# Autodesk Inventor assembly: wheel_axle
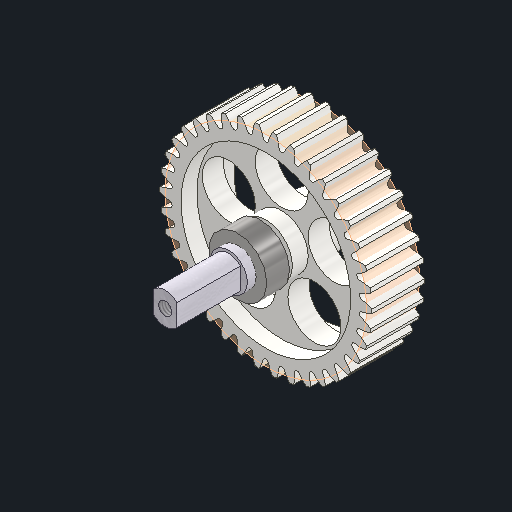
[picture p0: Inventor's stored thumbnail of the model, 512x512]
Saved by Autodesk Inventor 2023 (Build 270158000, 158)
## iProperties
Created: 2024-04-09
Part Number: wheel_axle
Document SubType Name: Assembly
Designer: szymo
Mass: 22 g
Surface Area: 67.2828 cm^2
Volume: 6.31995 cm^3
Density: 3.48104 g/cm^3
Author: szymo
## Documents named in this file (5)
- D:\roboilo\robots\codename wafel - australia\3d_parts\rev4\wheel_axle.iam
- D:\roboilo\robots\codename wafel - australia\3d_parts\rev4\MegaSumo kola zebate 38.ipt
- D:\roboilo\robots\codename wafel - australia\3d_parts\rev4\wal_kola.ipt
- D:\roboilo\robots\codename wafel - australia\3d_parts\rev4\small_bearing.ipt
- D:\roboilo\robots\codename wafel - australia\3d_parts\rev4\big_bearing.ipt
## Components (4 placed, 4 different names)
1. wal_kola:1 — Rotational:1, Flush:1, Flush:2
2. MegaSumo kola zebate 38:1 — Rotational:1
3. small_bearing:1 — Flush:1
4. big_bearing:1 — Flush:2
## Relationships (3: Flush 2, RevoluteJoint 1)
- Rotational:1 [RevoluteJoint]: wal_kola:1 ↔ MegaSumo kola zebate 38:1
- Flush:1: wal_kola:1 ↔ small_bearing:1
- Flush:2: wal_kola:1 ↔ big_bearing:1
